# Autodesk Inventor assembly: AM14U3 Long
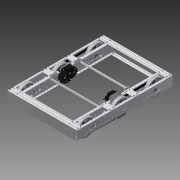
[picture p0: Inventor's stored thumbnail of the model, 180x180]
Saved by Autodesk Inventor 2016 SP1 (Build 200210100, 210)
## iProperties
Created: 2015-08-19
Part Number: AM14U3 Long
Description: STEP AP214
Document SubType Name: Assembly
Designer: PhillipD
Sending System: SolidWorks 2014
Preprocessor: SwSTEP 2.0
Title: AM14U3 Long.STEP
Revision Number: ANY
## Documents named in this file (2)
- D:\FIRST\FRC KOP 2016\FRC KOP 2016\Drive Base\DB_DriveBaseLong_AM14U3.iam
- D:\FIRST\FRC KOP 2016\FRC KOP 2016\Drive Base\Parts\AM14U3 Long Half.iam
## Components (2 placed, 2 different names)
1. AM14U3 Long Half_1 [sub-assembly] — Insert:1, Insert:2, Mate:1
2. AM14U3 Long Half_2 [sub-assembly] — Insert:1, Insert:2
## Relationships (3: Insert 2, Mate 1)
- Insert:1: AM14U3 Long Half_1 ↔ AM14U3 Long Half_2
- Insert:2: AM14U3 Long Half_1 ↔ AM14U3 Long Half_2
- Mate:1: AM14U3 Long Half_1
